# Autodesk Inventor assembly: Drive V3
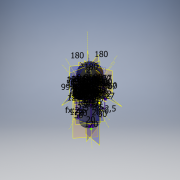
[picture p0: Inventor's stored thumbnail of the model, 180x180]
Saved by Autodesk Inventor 2019.1 (Build 231200000, 200)
## iProperties
Created: 2018-06-30
Part Number: Drive V3
Material: Generisch
Document SubType Name: Assembly
Designer: JochenAlt
Author: JochenAlt
## Documents named in this file (6)
- D:\Projects\Ondine\CAD\Drive V3.iam
- D:\Projects\Ondine\CAD\Sphere.ipt
- D:\Projects\Ondine\CAD\DriveChain V3.iam
- D:\Projects\Ondine\CAD\PCB\ControllerPCBHolder.ipt
- D:\Projects\Ondine\CAD\SpindleMotor.iam
- D:\Projects\Ondine\CAD\LegMotorHolder.ipt
## Components (7 placed, 5 different names)
1. Sphere:1 — Passend:38, Tangential:1
2. DriveChain V3:1 [sub-assembly] — Passend:41, Passend:47, Passend:56, Passend:57
3. DriveChain V3:2 [sub-assembly] — Passend:39, Tangential:1, Passend:46, Passend:55, Passend:56
4. DriveChain V3:3 [sub-assembly] — Passend:40, Passend:46, Passend:47, Passend:51, Winkel:1, Fluchtend:1, Fluchtend:2, Passend:55, Passend:58
5. PCBHolder:1 — Passend:57, Passend:58
6. SpindleMotor:1 [sub-assembly] — Fluchtend:1, Passend:52
7. LegMotorHolder:1 — Passend:51, Winkel:1, Fluchtend:2, Passend:52
## Relationships (16: Mate 12, Flush 2, Tangent 1, Angle 1)
- Passend:38 [Mate]: Sphere:1
- Passend:39 [Mate]: DriveChain V3:2
- Passend:40 [Mate]: DriveChain V3:3
- Passend:41 [Mate]: DriveChain V3:1
- Tangential:1: Sphere:1 ↔ DriveChain V3:2
- Passend:46 [Mate]: DriveChain V3:2 ↔ DriveChain V3:3
- Passend:47 [Mate]: DriveChain V3:1 ↔ DriveChain V3:3
- Passend:51 [Mate]: DriveChain V3:3 ↔ LegMotorHolder:1
- Winkel:1 [Angle] (180 deg): DriveChain V3:3 ↔ LegMotorHolder:1
- Fluchtend:1 [Flush]: DriveChain V3:3 ↔ SpindleMotor:1
- Fluchtend:2 [Flush]: DriveChain V3:3 ↔ LegMotorHolder:1
- Passend:52 [Mate]: SpindleMotor:1 ↔ LegMotorHolder:1
- Passend:55 [Mate]: DriveChain V3:2 ↔ DriveChain V3:3
- Passend:56 [Mate]: DriveChain V3:1 ↔ DriveChain V3:2
- Passend:57 [Mate]: DriveChain V3:1 ↔ PCBHolder:1
- Passend:58 [Mate]: DriveChain V3:3 ↔ PCBHolder:1
